# Autodesk Inventor assembly: FLUGGER FLOOR PAN
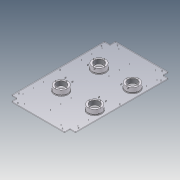
[picture p0: Inventor's stored thumbnail of the model, 180x180]
Saved by Autodesk Inventor 2020.3 (Build 243373000, 373)
## iProperties
RuleStatus: InUse
AfterDocSave0: file://Part Number Cleaner
Created: 2023-01-07
Catalog Web Link: https://www.janelia.org/
Vendor: HHMI: JRC - jET
Document SubType Name: Assembly
Designer: arnoldj
DESIGN DEPARTMENT: HHMI: JRC - jET
ALTERED ITEM PART NUMBER: N/A
ALTERED ITEM VENDOR: N/A
ALTERED ITEM DESCRIPTION: N/A
PART NUMBER - LEGACY: Standard
Author: arnoldj
Revision Number: 0
## Documents named in this file (4)
- C:\_WORKSPACE\DATA\PROJECTS\_PROJECTS BY LAB\CARD (LAB)\FLUGGER\FLUGGER FLOOR PAN.iam
- C:\_WORKSPACE\DATA\PROJECTS\_PROJECTS BY LAB\CARD (LAB)\FLUGGER\FLUGGER FLOOR PAN.ipt
- C:\_WORKSPACE\DATA\PROJECTS\_PROJECTS BY LAB\CARD (LAB)\FLUGGER\FLUGGER FLOOR CAP.ipt
- C:\_WORKSPACE\DATA\PROJECTS\_PROJECTS BY LAB\CARD (LAB)\FLUGGER\FLUGGER FLOOR WELL.ipt
## Components (9 placed, 3 different names)
1. FLUGGER FLOOR PAN:1 — Mate:1, Mate:5, Mate:6, Mate:7
2. FLUGGER FLOOR CAP:1 — Mate:1, Mate:5, Mate:6, Mate:8, Mate:9
3. FLUGGER FLOOR WELL:1 — Mate:7, Mate:8, Mate:9
4. FLUGGER FLOOR CAP:2
5. FLUGGER FLOOR WELL:2
6. FLUGGER FLOOR CAP:3
7. FLUGGER FLOOR WELL:3
8. FLUGGER FLOOR CAP:4
9. FLUGGER FLOOR WELL:4
## Component patterns: (4 elements, first: FLUGGER FLOOR CAP:1 + FLUGGER FLOOR WELL:1)
## Relationships (6: Mate 6)
- Mate:1 (31.75 mm): FLUGGER FLOOR PAN:1 ↔ FLUGGER FLOOR CAP:1
- Mate:5: FLUGGER FLOOR PAN:1 ↔ FLUGGER FLOOR CAP:1
- Mate:6: FLUGGER FLOOR PAN:1 ↔ FLUGGER FLOOR CAP:1
- Mate:7: FLUGGER FLOOR PAN:1 ↔ FLUGGER FLOOR WELL:1
- Mate:8: FLUGGER FLOOR CAP:1 ↔ FLUGGER FLOOR WELL:1
- Mate:9: FLUGGER FLOOR CAP:1 ↔ FLUGGER FLOOR WELL:1
